# Autodesk Inventor assembly: Section 3
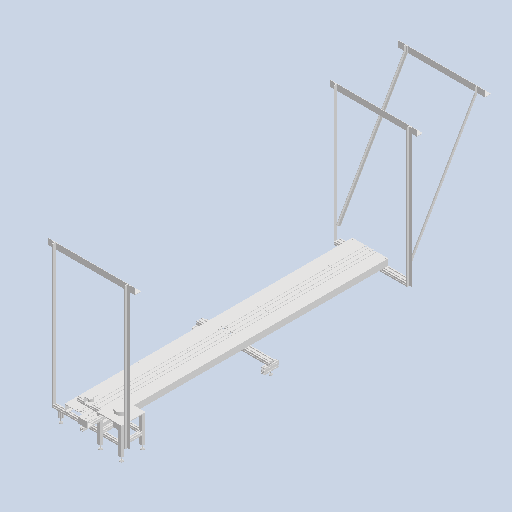
[picture p0: Inventor's stored thumbnail of the model, 512x512]
Saved by Autodesk Inventor 2023 (Build 270158030, 158C)
## iProperties
Created: 2022-07-14
Part Number: Section 3
Document SubType Name: Assembly
Designer: jeremyy
Author: jeremyy
## Documents named in this file (19)
- \\andrew.ad.cmu.edu\users\users1\jeremyy\Documents\Inventor\CMU Bridge\New folder\Section 3.iam
- \\andrew.ad.cmu.edu\users\users1\jeremyy\Documents\Inventor\CMU Bridge\New folder\LongC96.ipt
- \\andrew.ad.cmu.edu\users\users1\jeremyy\Documents\Inventor\CMU Bridge\New folder\LatXX24in.ipt
- \\andrew.ad.cmu.edu\users\users1\jeremyy\Documents\Inventor\CMU Bridge\New folder\LatX24in.ipt
- \\andrew.ad.cmu.edu\users\users1\jeremyy\Documents\Inventor\CMU Bridge\New folder\LongXX5.ipt
- \\andrew.ad.cmu.edu\users\users1\jeremyy\Documents\Inventor\CMU Bridge\New folder\VertL46in.ipt
- \\andrew.ad.cmu.edu\users\users1\jeremyy\Documents\Inventor\CMU Bridge\New folder\LatL29in.ipt
- \\andrew.ad.cmu.edu\users\users1\jeremyy\Documents\Inventor\CMU Bridge\New folder\VertX9in.ipt
- \\andrew.ad.cmu.edu\users\users1\jeremyy\Documents\Inventor\CMU Bridge\New folder\LatLongX6in.ipt
- \\andrew.ad.cmu.edu\users\users1\jeremyy\Documents\Inventor\CMU Bridge\New folder\Plate8inx8in.ipt
- \\andrew.ad.cmu.edu\users\users1\jeremyy\Documents\Inventor\CMU Bridge\New folder\VertL47.25in.ipt
- \\andrew.ad.cmu.edu\users\users1\jeremyy\Documents\Inventor\CMU Bridge\New folder\DiagL2.ipt
- \\andrew.ad.cmu.edu\users\users1\jeremyy\Documents\Inventor\CMU Bridge\New folder\DiagR2.ipt
- \\andrew.ad.cmu.edu\users\users1\jeremyy\Documents\Inventor\CMU Bridge\New folder\Motor.ipt
- \\andrew.ad.cmu.edu\users\users1\jeremyy\Documents\Inventor\CMU Bridge\New folder\Gear.iam
- \\andrew.ad.cmu.edu\users\users1\jeremyy\Documents\Inventor\CMU Bridge\New folder\Foot.ipt
- \\andrew.ad.cmu.edu\users\users1\jeremyy\Documents\Inventor\CMU Bridge\New folder\VertX2in.ipt
- \\andrew.ad.cmu.edu\users\users1\jeremyy\Documents\Inventor\CMU Bridge\New folder\Plate1ftx8ft.ipt
- \\andrew.ad.cmu.edu\users\users1\jeremyy\Documents\Inventor\CMU Bridge\New folder\PlateRailClamp48in.iam
## Components (42 placed, 18 different names)
1. LongC96:1 — Flush:5, Flush:6, Mate:5, Flush:9, Mate:45, Flush:59, Flush:60
2. LongC96:2 — Flush:5, Flush:6, Mate:4, Flush:7, Flush:8, Flush:10, Mate:6, Flush:11, Flush:12, Mate:45, Mate:46
3. LatXX24in:1 — Mate:4, Flush:7, Flush:8, Flush:16, Mate:13, Flush:23, Flush:24, Mate:14, Flush:25
4. LatX24in:1 — Mate:5, Flush:9, Flush:10, Mate:12, Flush:27, Mate:16, Flush:28, Mate:25, Flush:45, Flush:46, Mate:26, Flush:47, Flush:48, Mate:43, Flush:56
5. LatXX24in:2 — Mate:6, Flush:11, Flush:12, Mate:9, Flush:17, Flush:18, Mate:10, Flush:19, Flush:20
6. LongXX5:1 — Mate:13, Flush:23, Flush:24, Flush:26, Mate:36, Mate:37
7. LongXX5:2 — Flush:16, Mate:14, Flush:25, Mate:38, Tangent:2
8. VertL46in:1 — Mate:10, Flush:19, Flush:20, Mate:11, Flush:21, Flush:22, Mate:28, Flush:51
9. VertL46in:2 — Mate:9, Flush:17, Flush:18, Mate:30, Flush:52
10. LatL29in:1 — Mate:11, Flush:21, Flush:22, Mate:29, Mate:31, Flush:54
11. VertX9in:1 — Mate:12, Flush:26, Flush:27, Mate:15, Flush:30, Flush:34, Mate:24, Flush:43, Flush:44, Mate:39, Tangent:3
12. LatLongX6in:1 — Mate:15, Mate:16, Flush:28, Mate:17, Flush:29, Flush:32
13. VertX9in:2 — Mate:17, Flush:29, Flush:30, Mate:18, Flush:31, Mate:40, Tangent:4
14. LatLongX6in:2 — Mate:18, Flush:31, Flush:32, Mate:19, Flush:33, Flush:35
15. VertX9in:3 — Mate:19, Flush:33, Flush:34, Mate:20, Flush:36, Flush:37, Mate:41, Tangent:5
16. LatLongX6in:3 — Mate:20, Flush:35, Flush:36, Mate:21, Flush:38
17. VertX9in:4 — Mate:21, Flush:37, Flush:38, Mate:22, Flush:39, Flush:40, Mate:23, Mate:42, Tangent:6
18. VertX9in:5 — Mate:22, Flush:39, Flush:40, Flush:41, Flush:42, Mate:35, Flush:55
19. VertX9in:6 — Mate:23, Flush:41, Flush:42, Mate:34, Flush:58
20. Plate8inx8in:1 — Mate:24, Flush:43, Flush:44, Mate:33, Tangent:1
21. VertL47.25in:1 — Mate:25, Flush:45, Flush:46, Flush:49, Flush:50
22. VertL47.25in:2 — Mate:26, Flush:47, Flush:48, Mate:27, Flush:57
23. LatL29in:2 — Mate:27, Flush:49, Flush:50
24. DiagL2:1 — Mate:28, Flush:51, Mate:29
25. DiagR2:1 — Mate:30, Flush:52, Mate:31, Flush:53, Mate:32
26. LatL29in:3 — Flush:53, Mate:32, Flush:54
27. Motor:1 — Mate:33, Tangent:1
28. Gear:1 [sub-assembly] — Mate:34, Flush:58
29. Gear:2 [sub-assembly] — Mate:35, Flush:55
30. Foot:1 — Mate:36, Mate:37
31. Foot:2 — Mate:38, Tangent:2
32. Foot:3 — Mate:39, Tangent:3
33. Foot:4 — Mate:40, Tangent:4
34. Foot:5 — Mate:41, Tangent:5
35. Foot:6 — Mate:42, Tangent:6
36. VertX2in:1 — Mate:43, Flush:56, Flush:57, Mate:44, Tangent:7
37. Foot:7 — Mate:44, Tangent:7
38. Plate1ftx8ft:1 — Mate:46, Flush:59, Flush:60, Mate:47, Flush:61, Flush:62, Mate:48, Flush:63, Flush:64, Mate:49, Mate:51
39. PlateRailClamp48in:1 [sub-assembly] — Mate:47, Flush:61, Flush:62, Mate:52, Flush:66
40. PlateRailClamp48in:2 [sub-assembly] — Mate:48, Flush:63, Flush:64, Mate:50, Flush:65
41. PlateRailClamp48in:3 [sub-assembly] — Mate:49, Mate:50, Flush:65
42. PlateRailClamp48in:4 [sub-assembly] — Mate:51, Mate:52, Flush:66
## Relationships (113: Flush 59, Mate 47, Tangent 7)
- Flush:5: LongC96:1 ↔ LongC96:2
- Flush:6: LongC96:1 ↔ LongC96:2
- Mate:4: LongC96:2 ↔ LatXX24in:1
- Flush:7 (1219.2 mm): LongC96:2 ↔ LatXX24in:1
- Flush:8 (-203.2 mm): LongC96:2 ↔ LatXX24in:1
- Mate:5: LongC96:1 ↔ LatX24in:1
- Flush:9: LongC96:1 ↔ LatX24in:1
- Flush:10 (-203.2 mm): LongC96:2 ↔ LatX24in:1
- Mate:6: LongC96:2 ↔ LatXX24in:2
- Flush:11: LongC96:2 ↔ LatXX24in:2
- Flush:12 (-203.2 mm): LongC96:2 ↔ LatXX24in:2
- Flush:16 (-38.1 mm): LatXX24in:1 ↔ LongXX5:2
- Mate:9: LatXX24in:2 ↔ VertL46in:2
- Flush:17: LatXX24in:2 ↔ VertL46in:2
- Flush:18: LatXX24in:2 ↔ VertL46in:2
- Mate:10: LatXX24in:2 ↔ VertL46in:1
- Flush:19: LatXX24in:2 ↔ VertL46in:1
- Flush:20: LatXX24in:2 ↔ VertL46in:1
- Mate:11: VertL46in:1 ↔ LatL29in:1
- Flush:21: VertL46in:1 ↔ LatL29in:1
- Flush:22 (-38.1 mm): VertL46in:1 ↔ LatL29in:1
- Mate:12: LatX24in:1 ↔ VertX9in:1
- Mate:13: LatXX24in:1 ↔ LongXX5:1
- Flush:23: LatXX24in:1 ↔ LongXX5:1
- Flush:24 (-38.1 mm): LatXX24in:1 ↔ LongXX5:1
- Mate:14: LatXX24in:1 ↔ LongXX5:2
- Flush:25: LatXX24in:1 ↔ LongXX5:2
- Flush:26: LongXX5:1 ↔ VertX9in:1
- Flush:27: LatX24in:1 ↔ VertX9in:1
- Mate:15: VertX9in:1 ↔ LatLongX6in:1
- Mate:16: LatX24in:1 ↔ LatLongX6in:1
- Flush:28: LatX24in:1 ↔ LatLongX6in:1
- Mate:17: LatLongX6in:1 ↔ VertX9in:2
- Flush:29: LatLongX6in:1 ↔ VertX9in:2
- Flush:30: VertX9in:1 ↔ VertX9in:2
- Mate:18: VertX9in:2 ↔ LatLongX6in:2
- Flush:31: VertX9in:2 ↔ LatLongX6in:2
- Flush:32: LatLongX6in:1 ↔ LatLongX6in:2
- Mate:19: LatLongX6in:2 ↔ VertX9in:3
- Flush:33: LatLongX6in:2 ↔ VertX9in:3
- Flush:34: VertX9in:1 ↔ VertX9in:3
- Mate:20: VertX9in:3 ↔ LatLongX6in:3
- Flush:35: LatLongX6in:2 ↔ LatLongX6in:3
- Flush:36: VertX9in:3 ↔ LatLongX6in:3
- Mate:21: LatLongX6in:3 ↔ VertX9in:4
- Flush:37: VertX9in:3 ↔ VertX9in:4
- Flush:38: LatLongX6in:3 ↔ VertX9in:4
- Mate:22: VertX9in:4 ↔ VertX9in:5
- Flush:39: VertX9in:4 ↔ VertX9in:5
- Flush:40: VertX9in:4 ↔ VertX9in:5
- Mate:23: VertX9in:4 ↔ VertX9in:6
- Flush:41: VertX9in:5 ↔ VertX9in:6
- Flush:42: VertX9in:5 ↔ VertX9in:6
- Mate:24: VertX9in:1 ↔ Plate8inx8in:1
- Flush:43: VertX9in:1 ↔ Plate8inx8in:1
- Flush:44: VertX9in:1 ↔ Plate8inx8in:1
- Mate:25: LatX24in:1 ↔ VertL47.25in:1
- Flush:45: LatX24in:1 ↔ VertL47.25in:1
- Flush:46: LatX24in:1 ↔ VertL47.25in:1
- Mate:26: LatX24in:1 ↔ VertL47.25in:2
- Flush:47: LatX24in:1 ↔ VertL47.25in:2
- Flush:48: LatX24in:1 ↔ VertL47.25in:2
- Mate:27: VertL47.25in:2 ↔ LatL29in:2
- Flush:49 (-38.1 mm): VertL47.25in:1 ↔ LatL29in:2
- Flush:50: VertL47.25in:1 ↔ LatL29in:2
- Mate:28: VertL46in:1 ↔ DiagL2:1
- Flush:51: VertL46in:1 ↔ DiagL2:1
- Mate:29 (508 mm): LatL29in:1 ↔ DiagL2:1
- Mate:30: VertL46in:2 ↔ DiagR2:1
- Flush:52: VertL46in:2 ↔ DiagR2:1
- Mate:31 (508 mm): LatL29in:1 ↔ DiagR2:1
- Flush:53: DiagR2:1 ↔ LatL29in:3
- Mate:32: DiagR2:1 ↔ LatL29in:3
- Flush:54: LatL29in:1 ↔ LatL29in:3
- Mate:33: Plate8inx8in:1 ↔ Motor:1
- Tangent:1: Plate8inx8in:1 ↔ Motor:1
- Mate:34: VertX9in:6 ↔ Gear:1
- Mate:35: VertX9in:5 ↔ Gear:2
- Flush:55 (76.2 mm): VertX9in:5 ↔ Gear:2
- Mate:36: LongXX5:1 ↔ Foot:1
- Mate:37: LongXX5:1 ↔ Foot:1
- Mate:38: LongXX5:2 ↔ Foot:2
- Tangent:2: LongXX5:2 ↔ Foot:2
- Mate:39: VertX9in:1 ↔ Foot:3
- Tangent:3: VertX9in:1 ↔ Foot:3
- Mate:40: VertX9in:2 ↔ Foot:4
- Tangent:4: VertX9in:2 ↔ Foot:4
- Mate:41: VertX9in:3 ↔ Foot:5
- Tangent:5: VertX9in:3 ↔ Foot:5
- Mate:42: VertX9in:4 ↔ Foot:6
- Tangent:6: VertX9in:4 ↔ Foot:6
- Mate:43: LatX24in:1 ↔ VertX2in:1
- Flush:56: LatX24in:1 ↔ VertX2in:1
- Flush:57 (50.8 mm): VertL47.25in:2 ↔ VertX2in:1
- Mate:44: VertX2in:1 ↔ Foot:7
- Tangent:7: VertX2in:1 ↔ Foot:7
- Mate:45 (-304.8 mm): LongC96:1 ↔ LongC96:2
- Flush:58 (-25.4 mm): VertX9in:6 ↔ Gear:1
- Mate:46: LongC96:2 ↔ Plate1ftx8ft:1
- Flush:59: LongC96:1 ↔ Plate1ftx8ft:1
- Flush:60: LongC96:1 ↔ Plate1ftx8ft:1
- Mate:47: Plate1ftx8ft:1 ↔ PlateRailClamp48in:1
- Flush:61: Plate1ftx8ft:1 ↔ PlateRailClamp48in:1
- Flush:62 (95.25 mm): Plate1ftx8ft:1 ↔ PlateRailClamp48in:1
- Mate:48: Plate1ftx8ft:1 ↔ PlateRailClamp48in:2
- Flush:63: Plate1ftx8ft:1 ↔ PlateRailClamp48in:2
- Flush:64 (95.25 mm): Plate1ftx8ft:1 ↔ PlateRailClamp48in:2
- Mate:49: Plate1ftx8ft:1 ↔ PlateRailClamp48in:3
- Mate:50: PlateRailClamp48in:2 ↔ PlateRailClamp48in:3
- Flush:65: PlateRailClamp48in:2 ↔ PlateRailClamp48in:3
- Mate:51: Plate1ftx8ft:1 ↔ PlateRailClamp48in:4
- Mate:52: PlateRailClamp48in:1 ↔ PlateRailClamp48in:4
- Flush:66: PlateRailClamp48in:1 ↔ PlateRailClamp48in:4
